# Autodesk Inventor assembly: ASY MSC 900.3 base frame
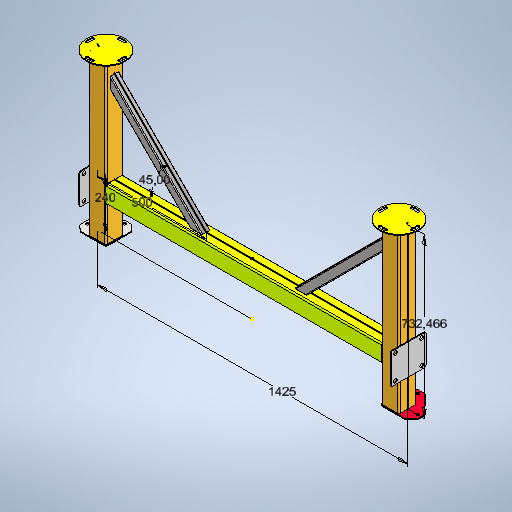
[picture p0: Inventor's stored thumbnail of the model, 512x512]
Saved by Autodesk Inventor 2025 (Build 290162010, 162A)
## iProperties
_SolveAssemblyDoc: Frame Generator Solve Assembly
_Version: 25.0.0
Created: 2024-06-27
Part Number: ASY MSC 900.3 base frame
Document SubType Name: Assembly
Designer: admin
Stock Number: ASY МОО 900.3 базовая рама
Author: admin
## Documents named in this file (7)
- C:\Users\pokla\Documents\Inventor\Отстойник осветлитель\Manturovo_Se-clar-Gleb\ASY MSC 900.3 base frame.iam
- C:\Users\pokla\Documents\Inventor\Отстойник осветлитель\Manturovo_Se-clar-Gleb\MSC DIM 009.3 base frame sketch.ipt
- C:\Users\pokla\Documents\Inventor\Отстойник осветлитель\Manturovo_Se-clar-Gleb\Pillars\ASY MSC 900.3.1 base frame.iam
- C:\Users\pokla\Documents\Inventor\Отстойник осветлитель\Manturovo_Se-clar-Gleb\MSC DIM 001 frame.ipt
- C:\Users\pokla\Documents\Inventor\Отстойник осветлитель\Manturovo_Se-clar-Gleb\MSC 906 flange frame.ipt
- C:\Users\pokla\Documents\Inventor\Отстойник осветлитель\Manturovo_Se-clar-Gleb\MSC 902 flange frame heel.ipt
- C:\Users\pokla\Documents\Inventor\Отстойник осветлитель\Manturovo_Se-clar-Gleb\MSC 908 transverse pillar plate.ipt
## Components (8 placed, 5 different names)
1. MSC DIM 009.3 base frame sketch:1 — Mate:1
2. ASY MSC 900.3.1 base frame:1 [sub-assembly] — Rigid:1, Rigid:2, Rigid:5, Rigid:6, Rigid:7, Rigid:8
3. MSC 906 flange frame:1 — Rigid:1
4. MSC 906 flange frame:2 — Rigid:2
5. MSC 902 flange frame heel:2 — Rigid:5
6. MSC 902 flange frame heel:3 — Rigid:6
7. MSC 908 transverse pillar plate:2 — Rigid:7
8. MSC 908 transverse pillar plate:3 — Rigid:8
## Relationships (7: WeldJoint 6, Mate 1)
- Rigid:1 [WeldJoint]: ASY MSC 900.3.1 base frame:1 ↔ MSC 906 flange frame:1
- Rigid:2 [WeldJoint]: ASY MSC 900.3.1 base frame:1 ↔ MSC 906 flange frame:2
- Mate:1: MSC DIM 009.3 base frame sketch:1
- Rigid:5 [WeldJoint]: ASY MSC 900.3.1 base frame:1 ↔ MSC 902 flange frame heel:2
- Rigid:6 [WeldJoint]: ASY MSC 900.3.1 base frame:1 ↔ MSC 902 flange frame heel:3
- Rigid:7 [WeldJoint] (80 mm): ASY MSC 900.3.1 base frame:1 ↔ MSC 908 transverse pillar plate:2
- Rigid:8 [WeldJoint] (80 mm): ASY MSC 900.3.1 base frame:1 ↔ MSC 908 transverse pillar plate:3
## Named parameters: frame_1 = 334.24956 mm, frame_3 = 2905.4 mm, frame_4 = 4190.97522 mm, frame_5 = 5476.55043 mm, Ширина_рамы = 1440 mm, Отступ_до_ниж_перекладины = 100 mm, Отступ_до_сред_перекладины = 1450 mm, Шаг_опор_по_баку = 2000 mm, Движение_рамы_вперед_назад = 270 mm, frame_2 = 1619.82478 mm, frame_6 = 6762.12565 mm
